# Autodesk Inventor assembly: mesoSPIM_excitation_path_MIR
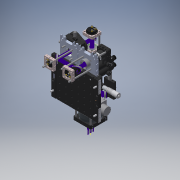
[picture p0: Inventor's stored thumbnail of the model, 180x180]
Saved by Autodesk Inventor 2016 (Build 200138000, 138)
## iProperties
Created: 2018-08-27
Part Number: mesoSPIM_excitation_path_MIR
Document SubType Name: Assembly
Designer: voigt
Author: voigt
## Documents named in this file (41)
- D:\Microscope_Design\CAD_Files\mesoSPIM_design\mesoSPIM\excitation_path\mesoSPIM_excitation_path_MIR.iam
- D:\Microscope_Design\CAD_Files\mesoSPIM_design\library\Thorlabs\large_area_translation_stages\tbb1515\TBB1515_M-Step_MIR.ipt
- D:\Microscope_Design\CAD_Files\mesoSPIM_design\mesoSPIM\excitation_path\components\Galvomount-22mm-diameter-Thorlabs-Right_MIR1.ipt
- D:\Microscope_Design\CAD_Files\mesoSPIM_design\library\Thorlabs\posts\1_inch_posts\RS2P_M_MIR2.ipt
- D:\Microscope_Design\CAD_Files\mesoSPIM_design\library\Thorlabs\posts\1_5_inch_post_spacers\PS5M_MIR.ipt
- D:\Microscope_Design\CAD_Files\mesoSPIM_design\library\Qioptiq\FLS40_rails\FLS40_150mm_MIR.ipt
- D:\Microscope_Design\CAD_Files\mesoSPIM_design\library\Thorlabs\30mm_cage_system\base_plates\CPVM-60mm_Baseplate_MIR.ipt
- D:\Microscope_Design\CAD_Files\mesoSPIM_design\library\Thorlabs\optics\AC254-075-A-ML-Step_MIR.ipt
- D:\Microscope_Design\CAD_Files\mesoSPIM_design\mesoSPIM\optical_design\cad_export_v1\mesoSPIM_excitation_path_optics_V1_MIR.iam
- D:\Microscope_Design\CAD_Files\mesoSPIM_design\library\Qioptiq\FLS40_carriers\FLS40_40mm_carrier_MIR.ipt
- D:\Microscope_Design\CAD_Files\mesoSPIM_design\library\Qioptiq\microbench\Cube_30_with35hole_MIR.ipt
- D:\Microscope_Design\CAD_Files\mesoSPIM_design\library\Qioptiq\microbench\Mounting_Plate_30_MIR.ipt
- D:\Microscope_Design\CAD_Files\mesoSPIM_design\mesoSPIM\excitation_path\components\fold_mirror_MIR.iam
- D:\Microscope_Design\CAD_Files\mesoSPIM_design\library\Qioptiq\FLS40_carriers\FLS40_20mm_carrier_MIR.ipt
- D:\Microscope_Design\CAD_Files\mesoSPIM_design\library\Qioptiq\microbench\Mounting_Plate_35_MIR.ipt
- D:\Microscope_Design\CAD_Files\mesoSPIM_design\library\Thorlabs\30mm_cage_system\cage_rods\ER3_CageRod.ipt
- D:\Microscope_Design\CAD_Files\Library_Files\Thorlabs\30mm_cage_system\rods\ER_CageRod.ipt
- D:\Microscope_Design\CAD_Files\mesoSPIM_design\library\Thorlabs\30mm_cage_system\xy_mount\ST1XY-S_M-Step_MIR.ipt
- D:\Microscope_Design\CAD_Files\mesoSPIM_design\library\Thorlabs\accessoires\SM1A39_Adapter_CmountExternal_SM1_External_MIR.ipt
- D:\Microscope_Design\CAD_Files\mesoSPIM_design\library\Optotune\EL-16-40\EL-16-40-TC-C (133-193-03-R0-01)_MIR.iam
- D:\Microscope_Design\CAD_Files\mesoSPIM_design\library\Thorlabs\30mm_cage_system\cage_rods\ER1_CageRod.ipt
- D:\Microscope_Design\CAD_Files\mesoSPIM_design\library\Thorlabs\30mm_cage_system\cage_rods\ER4_CageRod.ipt
- D:\Microscope_Design\CAD_Files\mesoSPIM_design\library\Thorlabs\30mm_cage_system\cage_rods\ER2_CageRod_MIR.ipt
- D:\Microscope_Design\CAD_Files\mesoSPIM_design\mesoSPIM\excitation_path\components\60mm-blank-cageplate-LCP03M-Nikon-MOD_MIR.ipt
- D:\Microscope_Design\CAD_Files\mesoSPIM_design\library\Thorlabs\other\F-Mount-AdapterSM2NFM-Step_MIR.ipt
- D:\Microscope_Design\CAD_Files\mesoSPIM_design\library\Nikon\50mm_1_4G_body_disassembled_MIR.ipt
- D:\Microscope_Design\CAD_Files\mesoSPIM_design\library\Thorlabs\accessoires\SM1FCA-APC-Fiberadapter_MIR.ipt
- D:\Microscope_Design\CAD_Files\mesoSPIM_design\library\Thorlabs\30mm_cage_system\cage_plates\SHCP025-Quarter-Inch-Shutter-Mount_MIR.ipt
- D:\Microscope_Design\CAD_Files\mesoSPIM_design\library\Thorlabs\30mm_cage_system\cage_plates\CP02_M_MIR.ipt
- D:\Microscope_Design\CAD_Files\mesoSPIM_design\library\Thorlabs\shutters\SHB025-Shutter_MIR.ipt
- D:\Microscope_Design\CAD_Files\mesoSPIM_design\library\Thorlabs\30mm_cage_system\SM1_tubes\SM1L10_MIR.ipt
- D:\Microscope_Design\CAD_Files\mesoSPIM_design\library\Thorlabs\30mm_cage_system\SM1_tubes\SM1V10_MIR.ipt
- D:\Microscope_Design\CAD_Files\mesoSPIM_design\library\Qioptiq\microbench\35mm_lens_mount\35mm Lens Mount_MIR.ipt
- D:\Microscope_Design\CAD_Files\mesoSPIM_design\library\Thorlabs\stages\XRN-B1_M-Micrometer-Baseplate_MIR.ipt
- D:\Microscope_Design\CAD_Files\mesoSPIM_design\library\Thorlabs\stages\XRN25C_M-25mm-Micrometer-Stage-Simplified_MIR.ipt
- D:\Microscope_Design\CAD_Files\mesoSPIM_design\library\Thorlabs\posts\post_mounts\PH75_M-Step_MIR.ipt
- D:\Microscope_Design\CAD_Files\mesoSPIM_design\library\Thorlabs\posts\12_7_mm_posts\TR50M_MIR.ipt
- D:\Microscope_Design\CAD_Files\mesoSPIM_design\library\Thorlabs\posts\12_7_mm_post_accessoires\RA180_M_MIR.ipt
- D:\Microscope_Design\CAD_Files\mesoSPIM_design\library\Qioptiq\microbench\Microbench_Holder_30_MIR.iam
- D:\Microscope_Design\CAD_Files\mesoSPIM_design\library\Thorlabs\posts\12_7_mm_posts\TR75M_MIR.ipt
- D:\Microscope_Design\CAD_Files\mesoSPIM_design\library\Thorlabs\galvos\GVS411_M_MIR.ipt
## Components (62 placed, 39 different names)
1. TBB1515_M-Step_MIR:1 — Mate:3, Mate:2, Mate:1, Flush:1, Mate:6, Mate:5, Mate:4, Mate:10, Mate:7, Mate:18, Mate:8, Mate:19, Mate:22, Mate:20, Mate:98, Mate:97, Mate:96
2. Galvomount-22mm-diameter-Thorlabs-Right_MIR1:1 — Mate:6, Mate:5, Mate:4, Flush:3, Mate:24, Mate:31, Flush:24, Mate:71, Mate:72, Mate:78, Angle:6, Angle:7, Angle:9, Mate:118, Mate:117
3. RS2P_M_MIR2:1 — Mate:10, Mate:7, Mate:12, Mate:11
4. RS2P_M_MIR2:2 — Mate:18, Mate:8, Mate:14, Mate:13
5. PS5M_MIR:1 — Mate:14, Mate:13, Mate:15, Mate:16
6. PS5M_MIR:2 — Mate:12, Mate:11, Mate:17
7. FLS40_150mm_MIR:1 — Flush:3, Mate:15, Flush:2, Flush:9, Mate:33, Mate:32, Mate:38, Mate:37
8. CPVM-60mm_Baseplate_MIR:1 — Mate:19, Mate:23, Flush:4, Mate:25, Mate:28, Mate:27, Flush:21, Mate:59, Flush:22, Mate:60, Mate:70, Flush:26, Mate:79, Flush:25, Mate:80, Mate:89, Mate:91, Mate:90
9. CPVM-60mm_Baseplate_MIR:2 — Mate:23, Flush:4, Mate:22, Mate:21, Mate:20, Mate:26, Mate:52, Angle:3, Mate:51, Mate:53, Mate:54, Flush:20, Mate:58, Flush:19, Mate:57, Mate:69
10. AC254-075-A-ML-Step_MIR:1 — Mate:28, Mate:27
11. mesoSPIM_excitation_path_optics_V1_MIR:1 [sub-assembly] — Mate:31, Mate:29
12. FLS40_40mm_carrier_MIR:1 — Flush:9, Mate:33, Mate:32, Flush:6, Flush:5, Mate:34
13. Cube_30_with35hole_MIR:1 — Flush:6, Flush:5, Mate:34, Flush:8, Mate:35, Flush:7, Flush:29, Mate:95, Flush:31
14. Mounting_Plate_30_MIR:1 — Flush:8, Mate:35, Flush:7, Angle:1, Flush:10, Mate:36
15. fold_mirror_MIR:1 [sub-assembly] — Angle:1, Flush:10, Mate:36
16. fold_mirror_MIR:2 [sub-assembly] — Mate:41, Mate:43, Angle:2
17. FLS40_20mm_carrier_MIR:1 — Mate:38, Mate:37, Flush:12, Flush:11, Mate:39
18. Mounting_Plate_35_MIR:1 — Flush:12, Flush:11, Mate:39, Mate:40, Flush:14, Flush:13, Flush:16, Flush:18, Flush:17
19. Mounting_Plate_35_MIR:2 — Mate:40, Flush:14, Flush:13, Mate:42, Mate:44, Flush:15, Mate:46, Flush:28, Mate:94
20. Mounting_Plate_30_MIR:2 — Mate:44, Mate:43, Angle:2, Flush:16, Flush:15, Mate:45
21. ER3_CageRod:1 — Flush:18, Mate:46
22. ER3_CageRod:2 — Flush:17, Mate:45
23. ST1XY-S_M-Step_MIR:1 — Mate:52, Angle:3, Mate:51, Mate:48, Mate:47, Mate:55, Mate:56
24. SM1A39_Adapter_CmountExternal_SM1_External_MIR:1 — Mate:48, Mate:47, Mate:50, Mate:49
25. EL-16-40-TC-C (133-193-03-R0-01)_MIR:1 [sub-assembly] — Mate:50, Mate:49
26. ER1_CageRod:3 — Mate:55, Mate:53
27. ER1_CageRod:4 — Mate:56, Mate:54
28. ER4_CageRod:5 — Flush:20, Mate:58, Mate:64
29. ER4_CageRod:6 — Flush:19, Mate:57, Mate:63
30. ER4_CageRod:7 — Flush:21, Mate:59, Mate:62
31. ER4_CageRod:8 — Flush:22, Mate:60, Mate:61
32. Mounting_Plate_30_MIR:3 — Mate:69, Mate:64, Mate:63, Angle:4, Mate:68, Mate:67
33. Mounting_Plate_30_MIR:4 — Mate:70, Mate:62, Mate:61, Angle:5, Mate:66, Mate:65
34. fold_mirror_MIR:3 [sub-assembly] — Angle:4, Mate:68, Mate:67
35. fold_mirror_MIR:4 [sub-assembly] — Angle:5, Mate:66, Mate:65
36. ER2_CageRod_MIR:1 — Flush:24, Mate:71, Flush:23, Mate:77
37. ER2_CageRod_MIR:2 — Flush:23, Mate:72
38. 60mm-blank-cageplate-LCP03M-Nikon-MOD_MIR:1 — Mate:78, Angle:6, Mate:77, Mate:74, Mate:73, Mate:76
39. F-Mount-AdapterSM2NFM-Step_MIR:1 — Mate:74, Mate:73, Mate:75
40. 50mm_1_4G_body_disassembled_MIR:1 — Mate:76, Mate:75
41. ER3_CageRod:9 — Flush:26, Mate:79, Mate:81, Mate:83
42. ER3_CageRod:10 — Flush:25, Mate:80, Mate:82, Mate:84
43. SM1FCA-APC-Fiberadapter_MIR:1 — Mate:88, Mate:87
44. SHCP025-Quarter-Inch-Shutter-Mount_MIR:1 — Mate:89, Mate:82, Mate:81, Mate:86, Flush:27, Mate:85, Mate:93
45. CP02_M_MIR:1 — Mate:88, Mate:86, Mate:84, Mate:83
46. SHB025-Shutter_MIR:1 — Mate:87, Flush:27, Mate:85
47. SM1L10_MIR:1 — Mate:91, Mate:90, Mate:92
48. SM1V10_MIR:1 — Mate:93, Mate:92
49. 35mm Lens Mount_MIR:1 — Flush:28, Mate:94
50. 35mm Lens Mount_MIR:2 — Flush:29, Mate:95
51. XRN-B1_M-Micrometer-Baseplate_MIR:1 — Mate:98, Mate:97, Mate:96, Flush:30, Mate:100, Mate:99
52. XRN25C_M-25mm-Micrometer-Stage-Simplified_MIR:1 — Flush:30, Mate:100, Mate:99, Mate:104, Mate:101, Mate:103, Mate:102
53. PH75_M-Step_MIR:1 — Mate:104, Mate:101, Mate:109
54. PH75_M-Step_MIR:2 — Mate:103, Mate:102, Mate:110, Mate:116
55. TR50M_MIR:1 — Mate:109, Mate:106, Mate:105
56. TR50M_MIR:2 — Mate:110, Mate:108, Mate:107
57. RA180_M_MIR:1 — Mate:106, Mate:105, Mate:111
58. RA180_M_MIR:2 — Mate:116, Mate:108, Mate:107, Mate:114
59. Microbench_Holder_30_MIR:1 [sub-assembly] — Flush:31, Angle:7, Mate:113, Mate:112, Flush:32, Angle:8, Mate:115
60. TR75M_MIR:1 — Mate:114, Mate:113, Mate:112, Mate:111
61. fold_mirror_MIR:5 [sub-assembly] — Flush:32, Angle:8, Mate:115
62. GVS411_M_MIR:1 — Angle:9, Mate:118, Mate:117
## Relationships (158: Mate 116, Flush 33, Angle 9)
- Mate:3 [Flush]: TBB1515_M-Step_MIR:1
- Mate:2: TBB1515_M-Step_MIR:1
- Mate:1: TBB1515_M-Step_MIR:1
- Flush:1 (40 mm): TBB1515_M-Step_MIR:1
- Mate:6: TBB1515_M-Step_MIR:1 ↔ Galvomount-22mm-diameter-Thorlabs-Right_MIR1:1
- Mate:5: TBB1515_M-Step_MIR:1 ↔ Galvomount-22mm-diameter-Thorlabs-Right_MIR1:1
- Mate:4: TBB1515_M-Step_MIR:1 ↔ Galvomount-22mm-diameter-Thorlabs-Right_MIR1:1
- Mate:10: TBB1515_M-Step_MIR:1 ↔ RS2P_M_MIR2:1
- Mate:7: TBB1515_M-Step_MIR:1 ↔ RS2P_M_MIR2:1
- Mate:18: TBB1515_M-Step_MIR:1 ↔ RS2P_M_MIR2:2
- Mate:8: TBB1515_M-Step_MIR:1 ↔ RS2P_M_MIR2:2
- Mate:14: RS2P_M_MIR2:2 ↔ PS5M_MIR:1
- Mate:13: RS2P_M_MIR2:2 ↔ PS5M_MIR:1
- Mate:12: RS2P_M_MIR2:1 ↔ PS5M_MIR:2
- Mate:11: RS2P_M_MIR2:1 ↔ PS5M_MIR:2
- Flush:3: Galvomount-22mm-diameter-Thorlabs-Right_MIR1:1 ↔ FLS40_150mm_MIR:1
- Mate:15: PS5M_MIR:1 ↔ FLS40_150mm_MIR:1
- Mate:17: PS5M_MIR:2
- Mate:16: PS5M_MIR:1
- Flush:2 (-20 mm): FLS40_150mm_MIR:1
- Mate:19: TBB1515_M-Step_MIR:1 ↔ CPVM-60mm_Baseplate_MIR:1
- Mate:23 (75 mm): CPVM-60mm_Baseplate_MIR:1 ↔ CPVM-60mm_Baseplate_MIR:2
- Flush:4: CPVM-60mm_Baseplate_MIR:1 ↔ CPVM-60mm_Baseplate_MIR:2
- Mate:22 (-2.98 mm): TBB1515_M-Step_MIR:1 ↔ CPVM-60mm_Baseplate_MIR:2
- Mate:21: CPVM-60mm_Baseplate_MIR:2
- Mate:20: TBB1515_M-Step_MIR:1 ↔ CPVM-60mm_Baseplate_MIR:2
- Mate:24: Galvomount-22mm-diameter-Thorlabs-Right_MIR1:1
- Mate:25: CPVM-60mm_Baseplate_MIR:1
- Mate:26: CPVM-60mm_Baseplate_MIR:2
- Mate:28: CPVM-60mm_Baseplate_MIR:1 ↔ AC254-075-A-ML-Step_MIR:1
- Mate:27: CPVM-60mm_Baseplate_MIR:1 ↔ AC254-075-A-ML-Step_MIR:1
- Mate:31: Galvomount-22mm-diameter-Thorlabs-Right_MIR1:1 ↔ mesoSPIM_excitation_path_optics_V1_MIR:1
- Mate:30
- Mate:29: mesoSPIM_excitation_path_optics_V1_MIR:1
- Flush:9: FLS40_150mm_MIR:1 ↔ FLS40_40mm_carrier_MIR:1
- Mate:33: FLS40_150mm_MIR:1 ↔ FLS40_40mm_carrier_MIR:1
- Mate:32: FLS40_150mm_MIR:1 ↔ FLS40_40mm_carrier_MIR:1
- Flush:6: FLS40_40mm_carrier_MIR:1 ↔ Cube_30_with35hole_MIR:1
- Flush:5: FLS40_40mm_carrier_MIR:1 ↔ Cube_30_with35hole_MIR:1
- Mate:34: FLS40_40mm_carrier_MIR:1 ↔ Cube_30_with35hole_MIR:1
- Flush:8: Cube_30_with35hole_MIR:1 ↔ Mounting_Plate_30_MIR:1
- Mate:35: Cube_30_with35hole_MIR:1 ↔ Mounting_Plate_30_MIR:1
- Flush:7: Cube_30_with35hole_MIR:1 ↔ Mounting_Plate_30_MIR:1
- Angle:1 (90 deg): Mounting_Plate_30_MIR:1 ↔ fold_mirror_MIR:1
- Flush:10 (-3.3 mm): Mounting_Plate_30_MIR:1 ↔ fold_mirror_MIR:1
- Mate:36: Mounting_Plate_30_MIR:1 ↔ fold_mirror_MIR:1
- Mate:38: FLS40_150mm_MIR:1 ↔ FLS40_20mm_carrier_MIR:1
- Mate:37: FLS40_150mm_MIR:1 ↔ FLS40_20mm_carrier_MIR:1
- Flush:12: FLS40_20mm_carrier_MIR:1 ↔ Mounting_Plate_35_MIR:1
- Flush:11: FLS40_20mm_carrier_MIR:1 ↔ Mounting_Plate_35_MIR:1
- Mate:39: FLS40_20mm_carrier_MIR:1 ↔ Mounting_Plate_35_MIR:1
- Mate:40 (3 mm): Mounting_Plate_35_MIR:1 ↔ Mounting_Plate_35_MIR:2
- Flush:14: Mounting_Plate_35_MIR:1 ↔ Mounting_Plate_35_MIR:2
- Flush:13: Mounting_Plate_35_MIR:1 ↔ Mounting_Plate_35_MIR:2
- Mate:42: Mounting_Plate_35_MIR:2
- Mate:41: fold_mirror_MIR:2
- Mate:44 (43.5 mm): Mounting_Plate_35_MIR:2 ↔ Mounting_Plate_30_MIR:2
- Mate:43: fold_mirror_MIR:2 ↔ Mounting_Plate_30_MIR:2
- Angle:2 (90 deg): fold_mirror_MIR:2 ↔ Mounting_Plate_30_MIR:2
- Flush:16: Mounting_Plate_35_MIR:1 ↔ Mounting_Plate_30_MIR:2
- Flush:15: Mounting_Plate_35_MIR:2 ↔ Mounting_Plate_30_MIR:2
- Flush:18: Mounting_Plate_35_MIR:1 ↔ ER3_CageRod:1
- Mate:46: Mounting_Plate_35_MIR:2 ↔ ER3_CageRod:1
- Flush:17: Mounting_Plate_35_MIR:1 ↔ ER3_CageRod:2
- Mate:45: Mounting_Plate_30_MIR:2 ↔ ER3_CageRod:2
- Mate:52 (2 mm): CPVM-60mm_Baseplate_MIR:2 ↔ ST1XY-S_M-Step_MIR:1
- Angle:3 (90 deg): CPVM-60mm_Baseplate_MIR:2 ↔ ST1XY-S_M-Step_MIR:1
- Mate:51: CPVM-60mm_Baseplate_MIR:2 ↔ ST1XY-S_M-Step_MIR:1
- Mate:48: ST1XY-S_M-Step_MIR:1 ↔ SM1A39_Adapter_CmountExternal_SM1_External_MIR:1
- Mate:47: ST1XY-S_M-Step_MIR:1 ↔ SM1A39_Adapter_CmountExternal_SM1_External_MIR:1
- Mate:50: SM1A39_Adapter_CmountExternal_SM1_External_MIR:1 ↔ EL-16-40-TC-C (133-193-03-R0-01)_MIR:1
- Mate:49: SM1A39_Adapter_CmountExternal_SM1_External_MIR:1 ↔ EL-16-40-TC-C (133-193-03-R0-01)_MIR:1
- Mate:55: ST1XY-S_M-Step_MIR:1 ↔ ER1_CageRod:3
- Mate:53: CPVM-60mm_Baseplate_MIR:2 ↔ ER1_CageRod:3
- Mate:56: ST1XY-S_M-Step_MIR:1 ↔ ER1_CageRod:4
- Mate:54: CPVM-60mm_Baseplate_MIR:2 ↔ ER1_CageRod:4
- Flush:20: CPVM-60mm_Baseplate_MIR:2 ↔ ER4_CageRod:5
- Mate:58: CPVM-60mm_Baseplate_MIR:2 ↔ ER4_CageRod:5
- Flush:19: CPVM-60mm_Baseplate_MIR:2 ↔ ER4_CageRod:6
- Mate:57: CPVM-60mm_Baseplate_MIR:2 ↔ ER4_CageRod:6
- Flush:21: CPVM-60mm_Baseplate_MIR:1 ↔ ER4_CageRod:7
- Mate:59: CPVM-60mm_Baseplate_MIR:1 ↔ ER4_CageRod:7
- Flush:22: CPVM-60mm_Baseplate_MIR:1 ↔ ER4_CageRod:8
- Mate:60: CPVM-60mm_Baseplate_MIR:1 ↔ ER4_CageRod:8
- Mate:69 (71 mm): CPVM-60mm_Baseplate_MIR:2 ↔ Mounting_Plate_30_MIR:3
- Mate:64: ER4_CageRod:5 ↔ Mounting_Plate_30_MIR:3
- Mate:63: ER4_CageRod:6 ↔ Mounting_Plate_30_MIR:3
- Mate:70 (71 mm): CPVM-60mm_Baseplate_MIR:1 ↔ Mounting_Plate_30_MIR:4
- Mate:62: ER4_CageRod:7 ↔ Mounting_Plate_30_MIR:4
- Mate:61: ER4_CageRod:8 ↔ Mounting_Plate_30_MIR:4
- Angle:4 (0 deg): Mounting_Plate_30_MIR:3 ↔ fold_mirror_MIR:3
- Mate:68: Mounting_Plate_30_MIR:3 ↔ fold_mirror_MIR:3
- Mate:67: Mounting_Plate_30_MIR:3 ↔ fold_mirror_MIR:3
- Angle:5 (0 deg): Mounting_Plate_30_MIR:4 ↔ fold_mirror_MIR:4
- Mate:66: Mounting_Plate_30_MIR:4 ↔ fold_mirror_MIR:4
- Mate:65: Mounting_Plate_30_MIR:4 ↔ fold_mirror_MIR:4
- Flush:24 (42 mm): Galvomount-22mm-diameter-Thorlabs-Right_MIR1:1 ↔ ER2_CageRod_MIR:1
- Mate:71: Galvomount-22mm-diameter-Thorlabs-Right_MIR1:1 ↔ ER2_CageRod_MIR:1
- Flush:23: ER2_CageRod_MIR:1 ↔ ER2_CageRod_MIR:2
- Mate:72: Galvomount-22mm-diameter-Thorlabs-Right_MIR1:1 ↔ ER2_CageRod_MIR:2
- Mate:78 (30 mm): Galvomount-22mm-diameter-Thorlabs-Right_MIR1:1 ↔ 60mm-blank-cageplate-LCP03M-Nikon-MOD_MIR:1
- Angle:6 (0 deg): Galvomount-22mm-diameter-Thorlabs-Right_MIR1:1 ↔ 60mm-blank-cageplate-LCP03M-Nikon-MOD_MIR:1
- Mate:77: ER2_CageRod_MIR:1 ↔ 60mm-blank-cageplate-LCP03M-Nikon-MOD_MIR:1
- Mate:74: 60mm-blank-cageplate-LCP03M-Nikon-MOD_MIR:1 ↔ F-Mount-AdapterSM2NFM-Step_MIR:1
- Mate:73: 60mm-blank-cageplate-LCP03M-Nikon-MOD_MIR:1 ↔ F-Mount-AdapterSM2NFM-Step_MIR:1
- Mate:76: 60mm-blank-cageplate-LCP03M-Nikon-MOD_MIR:1 ↔ 50mm_1_4G_body_disassembled_MIR:1
- Mate:75: F-Mount-AdapterSM2NFM-Step_MIR:1 ↔ 50mm_1_4G_body_disassembled_MIR:1
- Flush:26: CPVM-60mm_Baseplate_MIR:1 ↔ ER3_CageRod:9
- Mate:79: CPVM-60mm_Baseplate_MIR:1 ↔ ER3_CageRod:9
- Flush:25: CPVM-60mm_Baseplate_MIR:1 ↔ ER3_CageRod:10
- Mate:80: CPVM-60mm_Baseplate_MIR:1 ↔ ER3_CageRod:10
- Mate:89 (48.9 mm): CPVM-60mm_Baseplate_MIR:1 ↔ SHCP025-Quarter-Inch-Shutter-Mount_MIR:1
- Mate:82: ER3_CageRod:10 ↔ SHCP025-Quarter-Inch-Shutter-Mount_MIR:1
- Mate:81: ER3_CageRod:9 ↔ SHCP025-Quarter-Inch-Shutter-Mount_MIR:1
- Mate:88: SM1FCA-APC-Fiberadapter_MIR:1 ↔ CP02_M_MIR:1
- Mate:86: SHCP025-Quarter-Inch-Shutter-Mount_MIR:1 ↔ CP02_M_MIR:1
- Mate:84: ER3_CageRod:10 ↔ CP02_M_MIR:1
- Mate:83: ER3_CageRod:9 ↔ CP02_M_MIR:1
- Mate:87: SM1FCA-APC-Fiberadapter_MIR:1 ↔ SHB025-Shutter_MIR:1
- Flush:27: SHCP025-Quarter-Inch-Shutter-Mount_MIR:1 ↔ SHB025-Shutter_MIR:1
- Mate:85: SHCP025-Quarter-Inch-Shutter-Mount_MIR:1 ↔ SHB025-Shutter_MIR:1
- Mate:91: CPVM-60mm_Baseplate_MIR:1 ↔ SM1L10_MIR:1
- Mate:90: CPVM-60mm_Baseplate_MIR:1 ↔ SM1L10_MIR:1
- Mate:93: SHCP025-Quarter-Inch-Shutter-Mount_MIR:1 ↔ SM1V10_MIR:1
- Mate:92: SM1L10_MIR:1 ↔ SM1V10_MIR:1
- Flush:28 (-0.6 mm): Mounting_Plate_35_MIR:2 ↔ 35mm Lens Mount_MIR:1
- Mate:94: Mounting_Plate_35_MIR:2 ↔ 35mm Lens Mount_MIR:1
- Flush:29 (8.45 mm): Cube_30_with35hole_MIR:1 ↔ 35mm Lens Mount_MIR:2
- Mate:95: Cube_30_with35hole_MIR:1 ↔ 35mm Lens Mount_MIR:2
- Mate:98: TBB1515_M-Step_MIR:1 ↔ XRN-B1_M-Micrometer-Baseplate_MIR:1
- Mate:97: TBB1515_M-Step_MIR:1 ↔ XRN-B1_M-Micrometer-Baseplate_MIR:1
- Mate:96: TBB1515_M-Step_MIR:1 ↔ XRN-B1_M-Micrometer-Baseplate_MIR:1
- Flush:30: XRN-B1_M-Micrometer-Baseplate_MIR:1 ↔ XRN25C_M-25mm-Micrometer-Stage-Simplified_MIR:1
- Mate:100: XRN-B1_M-Micrometer-Baseplate_MIR:1 ↔ XRN25C_M-25mm-Micrometer-Stage-Simplified_MIR:1
- Mate:99: XRN-B1_M-Micrometer-Baseplate_MIR:1 ↔ XRN25C_M-25mm-Micrometer-Stage-Simplified_MIR:1
- Mate:104: XRN25C_M-25mm-Micrometer-Stage-Simplified_MIR:1 ↔ PH75_M-Step_MIR:1
- Mate:101: XRN25C_M-25mm-Micrometer-Stage-Simplified_MIR:1 ↔ PH75_M-Step_MIR:1
- Mate:103: XRN25C_M-25mm-Micrometer-Stage-Simplified_MIR:1 ↔ PH75_M-Step_MIR:2
- Mate:102: XRN25C_M-25mm-Micrometer-Stage-Simplified_MIR:1 ↔ PH75_M-Step_MIR:2
- Mate:109: PH75_M-Step_MIR:1 ↔ TR50M_MIR:1
- Mate:110: PH75_M-Step_MIR:2 ↔ TR50M_MIR:2
- Mate:106: TR50M_MIR:1 ↔ RA180_M_MIR:1
- Mate:105: TR50M_MIR:1 ↔ RA180_M_MIR:1
- Mate:116: PH75_M-Step_MIR:2 ↔ RA180_M_MIR:2
- Mate:108: TR50M_MIR:2 ↔ RA180_M_MIR:2
- Mate:107: TR50M_MIR:2 ↔ RA180_M_MIR:2
- Flush:31: Cube_30_with35hole_MIR:1 ↔ Microbench_Holder_30_MIR:1
- Angle:7 (0 deg): Galvomount-22mm-diameter-Thorlabs-Right_MIR1:1 ↔ Microbench_Holder_30_MIR:1
- Mate:114: RA180_M_MIR:2 ↔ TR75M_MIR:1
- Mate:113: Microbench_Holder_30_MIR:1 ↔ TR75M_MIR:1
- Mate:112: Microbench_Holder_30_MIR:1 ↔ TR75M_MIR:1
- Mate:111: RA180_M_MIR:1 ↔ TR75M_MIR:1
- Flush:32 (4.4 mm): Microbench_Holder_30_MIR:1 ↔ fold_mirror_MIR:5
- Angle:8 (0 deg): Microbench_Holder_30_MIR:1 ↔ fold_mirror_MIR:5
- Mate:115: Microbench_Holder_30_MIR:1 ↔ fold_mirror_MIR:5
- Angle:9 (45 deg): Galvomount-22mm-diameter-Thorlabs-Right_MIR1:1 ↔ GVS411_M_MIR:1
- Mate:118: Galvomount-22mm-diameter-Thorlabs-Right_MIR1:1 ↔ GVS411_M_MIR:1
- Mate:117: Galvomount-22mm-diameter-Thorlabs-Right_MIR1:1 ↔ GVS411_M_MIR:1
